# Autodesk Inventor assembly: robot_arm
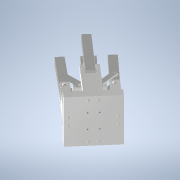
[picture p0: Inventor's stored thumbnail of the model, 180x180]
Saved by Autodesk Inventor 2021 (Build 250183000, 183)
## iProperties
Created: 2021-10-07
Part Number: robot_arm
Document SubType Name: Assembly
Designer: ryusei
Author: ryusei
## Documents named in this file (13)
- C:\Users\ryusei\Documents\Inventor\robot_design3\試作品1号\robot_arm.iam
- C:\Users\ryusei\Documents\Inventor\robot_design3\試作品1号\部品\土台.ipt
- C:\Users\ryusei\Documents\Inventor\robot_design3\試作品1号\部品\アーム支え.ipt
- C:\Users\ryusei\Documents\Inventor\robot_design3\試作品1号\部品\MF63ZZ_ベアリング.ipt
- C:\Users\ryusei\Documents\Inventor\robot_design3\試作品1号\部品\ステンレス平行ピンΦ3h7_20.ipt
- C:\Users\ryusei\Documents\Inventor\robot_design3\試作品1号\部品\シリンダ固定.ipt
- C:\Users\ryusei\Documents\Inventor\robot_design3\試作品1号\部品\シリンダ先端パーツ.ipt
- C:\Users\ryusei\Documents\Inventor\robot_design3\試作品1号\部品\アーム10×10×60.ipt
- C:\Users\ryusei\Documents\Inventor\robot_design3\試作品1号\部品\ステンレス平行ピンΦ3h7_16.ipt
- C:\Users\ryusei\Documents\Inventor\robot_design3\試作品1号\MBDA6×15_シリンダコガネイ\伸びるやつ１.ipt
- C:\Users\ryusei\Documents\Inventor\robot_design3\試作品1号\MBDA6×15_シリンダコガネイ\伸びるやつ2.ipt
- C:\Users\ryusei\Documents\Inventor\robot_design3\試作品1号\MBDA6×15_シリンダコガネイ\本体.ipt
- C:\Users\ryusei\Documents\Inventor\robot_design3\試作品1号\部品\リンク26×6×2.ipt
## Components (59 placed, 12 different names)
1. 土台:1 — 挿入:17, 挿入:18, 挿入:21, 挿入:22, 角度:1, 挿入:56, 挿入:57, 挿入:58, 挿入:59, 挿入:60, 挿入:61, 挿入:62, 挿入:63, 挿入:64, 挿入:65, 挿入:66, 挿入:67, 挿入:68, 挿入:69, 挿入:70, 挿入:71, 挿入:72, 挿入:73
2. アーム支え:1 — 挿入:9, 挿入:10, 挿入:62, 挿入:63, 挿入:72, 挿入:73
3. アーム支え:2 — 挿入:11, 挿入:12, 挿入:56, 挿入:57, 挿入:60, 挿入:61, 挿入:66, 挿入:67
4. アーム支え:3 — 挿入:13, 挿入:14, 挿入:58, 挿入:59, 挿入:68, 挿入:69
5. アーム支え:4 — 挿入:15, 挿入:16, 挿入:64, 挿入:65, 挿入:70, 挿入:71
6. MF63ZZ_ベアリング:1 — 挿入:15
7. MF63ZZ_ベアリング:2 — 挿入:13, メイト:3
8. MF63ZZ_ベアリング:3 — 挿入:10
9. MF63ZZ_ベアリング:4 — 挿入:12
10. MF63ZZ_ベアリング:5 — 挿入:16, メイト:18
11. MF63ZZ_ベアリング:6 — 挿入:11, メイト:4
12. MF63ZZ_ベアリング:7 — 挿入:14
13. MF63ZZ_ベアリング:8 — 挿入:9, メイト:2
14. ステンレス平行ピンΦ3h7_20:1 — メイト:4, メイト:8
15. ステンレス平行ピンΦ3h7_20:2 — メイト:3, メイト:5
16. ステンレス平行ピンΦ3h7_20:3 — メイト:2, メイト:7
17. シリンダ固定:1 — 挿入:17, 挿入:18
18. シリンダ固定:2 — 挿入:21, 挿入:22, 挿入:44, 挿入:45
19. アーム10×10×60:1 — メイト:8, 挿入:40, 挿入:41
20. アーム10×10×60:2 — メイト:7, 挿入:34, 挿入:35
21. アーム10×10×60:3 — メイト:5, 挿入:38, 挿入:39
22. アーム10×10×60:4 — 挿入:36, 挿入:37, メイト:19
23. MF63ZZ_ベアリング:17 — 挿入:40, メイト:12
24. MF63ZZ_ベアリング:18 — 挿入:41
25. MF63ZZ_ベアリング:19 — 挿入:36, メイト:9
26. MF63ZZ_ベアリング:20 — 挿入:37
27. MF63ZZ_ベアリング:21 — 挿入:38, メイト:10
28. MF63ZZ_ベアリング:22 — 挿入:39
29. MF63ZZ_ベアリング:23 — 挿入:35
30. MF63ZZ_ベアリング:24 — 挿入:34, メイト:11
31. ステンレス平行ピンΦ3h7_16:3 — メイト:12, 挿入:86, 挿入:99
32. ステンレス平行ピンΦ3h7_16:5 — メイト:11, 挿入:96, 挿入:101
33. ステンレス平行ピンΦ3h7_16:6 — メイト:9, 挿入:93, 挿入:95
34. ステンレス平行ピンΦ3h7_16:7 — メイト:10, 挿入:89, 挿入:91
35. シリンダ先端パーツ:1 — 角度:1, 挿入:46, 挿入:47, 挿入:48, 挿入:49, 挿入:50, 挿入:51, 挿入:52, 挿入:53
36. 伸びるやつ１:1
37. 伸びるやつ2:1
38. 本体:1 — 挿入:44, 挿入:45
39. MF63ZZ_ベアリング:25 — 挿入:49, メイト:14
40. MF63ZZ_ベアリング:26 — 挿入:48
41. MF63ZZ_ベアリング:27 — 挿入:47
42. MF63ZZ_ベアリング:28 — 挿入:46, メイト:16
43. MF63ZZ_ベアリング:29 — 挿入:50, メイト:15
44. MF63ZZ_ベアリング:30 — 挿入:51
45. MF63ZZ_ベアリング:31 — 挿入:52, メイト:17
46. MF63ZZ_ベアリング:32 — 挿入:53
47. ステンレス平行ピンΦ3h7_16:8 — メイト:16, 挿入:97, 挿入:100
48. ステンレス平行ピンΦ3h7_16:9 — メイト:15, 挿入:88, 挿入:90
49. ステンレス平行ピンΦ3h7_16:11 — メイト:14, 挿入:87, 挿入:98
50. ステンレス平行ピンΦ3h7_16:12 — メイト:17, 挿入:92, 挿入:94
51. ステンレス平行ピンΦ3h7_20:4 — メイト:18, メイト:19
52. リンク26×6×2:1 — 挿入:92, 挿入:93
53. リンク26×6×2:2 — 挿入:100, 挿入:101
54. リンク26×6×2:3 — 挿入:98, 挿入:99
55. リンク26×6×2:4 — 挿入:96, 挿入:97
56. リンク26×6×2:5 — 挿入:94, 挿入:95
57. リンク26×6×2:6 — 挿入:90, 挿入:91
58. リンク26×6×2:7 — 挿入:88, 挿入:89
59. リンク26×6×2:8 — 挿入:86, 挿入:87
## Relationships (84: Insert 66, Mate 17, Angle 1)
- 挿入:9 [Insert]: アーム支え:1 ↔ MF63ZZ_ベアリング:8
- 挿入:10 [Insert]: アーム支え:1 ↔ MF63ZZ_ベアリング:3
- 挿入:11 [Insert]: アーム支え:2 ↔ MF63ZZ_ベアリング:6
- 挿入:12 [Insert]: アーム支え:2 ↔ MF63ZZ_ベアリング:4
- 挿入:13 [Insert]: アーム支え:3 ↔ MF63ZZ_ベアリング:2
- 挿入:14 [Insert]: アーム支え:3 ↔ MF63ZZ_ベアリング:7
- 挿入:15 [Insert]: アーム支え:4 ↔ MF63ZZ_ベアリング:1
- 挿入:16 [Insert]: アーム支え:4 ↔ MF63ZZ_ベアリング:5
- メイト:2 [Mate]: MF63ZZ_ベアリング:8 ↔ ステンレス平行ピンΦ3h7_20:3
- メイト:3 [Mate]: MF63ZZ_ベアリング:2 ↔ ステンレス平行ピンΦ3h7_20:2
- メイト:4 [Mate]: MF63ZZ_ベアリング:6 ↔ ステンレス平行ピンΦ3h7_20:1
- 挿入:17 [Insert]: 土台:1 ↔ シリンダ固定:1
- 挿入:18 [Insert]: 土台:1 ↔ シリンダ固定:1
- 挿入:21 [Insert]: 土台:1 ↔ シリンダ固定:2
- 挿入:22 [Insert]: 土台:1 ↔ シリンダ固定:2
- メイト:5 [Mate]: ステンレス平行ピンΦ3h7_20:2 ↔ アーム10×10×60:3
- メイト:7 [Mate]: ステンレス平行ピンΦ3h7_20:3 ↔ アーム10×10×60:2
- メイト:8 [Mate]: ステンレス平行ピンΦ3h7_20:1 ↔ アーム10×10×60:1
- 挿入:34 [Insert]: アーム10×10×60:2 ↔ MF63ZZ_ベアリング:24
- 挿入:35 [Insert]: アーム10×10×60:2 ↔ MF63ZZ_ベアリング:23
- 挿入:36 [Insert]: アーム10×10×60:4 ↔ MF63ZZ_ベアリング:19
- 挿入:37 [Insert]: アーム10×10×60:4 ↔ MF63ZZ_ベアリング:20
- 挿入:38 [Insert]: アーム10×10×60:3 ↔ MF63ZZ_ベアリング:21
- 挿入:39 [Insert]: アーム10×10×60:3 ↔ MF63ZZ_ベアリング:22
- 挿入:40 [Insert]: アーム10×10×60:1 ↔ MF63ZZ_ベアリング:17
- 挿入:41 [Insert]: アーム10×10×60:1 ↔ MF63ZZ_ベアリング:18
- メイト:9 [Mate]: MF63ZZ_ベアリング:19 ↔ ステンレス平行ピンΦ3h7_16:6
- メイト:10 [Mate]: MF63ZZ_ベアリング:21 ↔ ステンレス平行ピンΦ3h7_16:7
- メイト:11 [Mate]: MF63ZZ_ベアリング:24 ↔ ステンレス平行ピンΦ3h7_16:5
- メイト:12 [Mate]: MF63ZZ_ベアリング:17 ↔ ステンレス平行ピンΦ3h7_16:3
- [Insert]: 伸びるやつ１:1 ↔ 伸びるやつ2:1
- [Mate]: 伸びるやつ１:1 ↔ 本体:1
- [Insert]: シリンダ先端パーツ:1 ↔ 伸びるやつ１:1
- 挿入:44 [Insert]: シリンダ固定:2 ↔ 本体:1
- 挿入:45 [Insert]: シリンダ固定:2 ↔ 本体:1
- 角度:1 [Angle] (0 deg): 土台:1 ↔ シリンダ先端パーツ:1
- 挿入:46 [Insert]: シリンダ先端パーツ:1 ↔ MF63ZZ_ベアリング:28
- 挿入:47 [Insert]: シリンダ先端パーツ:1 ↔ MF63ZZ_ベアリング:27
- 挿入:48 [Insert]: シリンダ先端パーツ:1 ↔ MF63ZZ_ベアリング:26
- 挿入:49 [Insert]: シリンダ先端パーツ:1 ↔ MF63ZZ_ベアリング:25
- 挿入:50 [Insert]: シリンダ先端パーツ:1 ↔ MF63ZZ_ベアリング:29
- 挿入:51 [Insert]: シリンダ先端パーツ:1 ↔ MF63ZZ_ベアリング:30
- 挿入:52 [Insert]: シリンダ先端パーツ:1 ↔ MF63ZZ_ベアリング:31
- 挿入:53 [Insert]: シリンダ先端パーツ:1 ↔ MF63ZZ_ベアリング:32
- メイト:14 [Mate]: MF63ZZ_ベアリング:25 ↔ ステンレス平行ピンΦ3h7_16:11
- メイト:15 [Mate]: MF63ZZ_ベアリング:29 ↔ ステンレス平行ピンΦ3h7_16:9
- メイト:16 [Mate]: MF63ZZ_ベアリング:28 ↔ ステンレス平行ピンΦ3h7_16:8
- メイト:17 [Mate]: MF63ZZ_ベアリング:31 ↔ ステンレス平行ピンΦ3h7_16:12
- 挿入:56 [Insert]: 土台:1 ↔ アーム支え:2
- 挿入:57 [Insert]: 土台:1 ↔ アーム支え:2
- 挿入:58 [Insert]: 土台:1 ↔ アーム支え:3
- 挿入:59 [Insert]: 土台:1 ↔ アーム支え:3
- 挿入:60 [Insert]: 土台:1 ↔ アーム支え:2
- 挿入:61 [Insert]: 土台:1 ↔ アーム支え:2
- 挿入:62 [Insert]: 土台:1 ↔ アーム支え:1
- 挿入:63 [Insert]: 土台:1 ↔ アーム支え:1
- 挿入:64 [Insert]: 土台:1 ↔ アーム支え:4
- 挿入:65 [Insert]: 土台:1 ↔ アーム支え:4
- 挿入:66 [Insert]: 土台:1 ↔ アーム支え:2
- 挿入:67 [Insert]: 土台:1 ↔ アーム支え:2
- 挿入:68 [Insert]: 土台:1 ↔ アーム支え:3
- 挿入:69 [Insert]: 土台:1 ↔ アーム支え:3
- 挿入:70 [Insert]: 土台:1 ↔ アーム支え:4
- 挿入:71 [Insert]: 土台:1 ↔ アーム支え:4
- 挿入:72 [Insert]: 土台:1 ↔ アーム支え:1
- 挿入:73 [Insert]: 土台:1 ↔ アーム支え:1
- メイト:18 [Mate]: MF63ZZ_ベアリング:5 ↔ ステンレス平行ピンΦ3h7_20:4
- メイト:19 [Mate]: アーム10×10×60:4 ↔ ステンレス平行ピンΦ3h7_20:4
- 挿入:86 [Insert]: ステンレス平行ピンΦ3h7_16:3 ↔ リンク26×6×2:8
- 挿入:87 [Insert]: ステンレス平行ピンΦ3h7_16:11 ↔ リンク26×6×2:8
- 挿入:88 [Insert]: ステンレス平行ピンΦ3h7_16:9 ↔ リンク26×6×2:7
- 挿入:89 [Insert]: ステンレス平行ピンΦ3h7_16:7 ↔ リンク26×6×2:7
- 挿入:90 [Insert]: ステンレス平行ピンΦ3h7_16:9 ↔ リンク26×6×2:6
- 挿入:91 [Insert]: ステンレス平行ピンΦ3h7_16:7 ↔ リンク26×6×2:6
- 挿入:92 [Insert]: ステンレス平行ピンΦ3h7_16:12 ↔ リンク26×6×2:1
- 挿入:93 [Insert]: ステンレス平行ピンΦ3h7_16:6 ↔ リンク26×6×2:1
- 挿入:94 [Insert]: ステンレス平行ピンΦ3h7_16:12 ↔ リンク26×6×2:5
- 挿入:95 [Insert]: ステンレス平行ピンΦ3h7_16:6 ↔ リンク26×6×2:5
- 挿入:96 [Insert]: ステンレス平行ピンΦ3h7_16:5 ↔ リンク26×6×2:4
- 挿入:97 [Insert]: ステンレス平行ピンΦ3h7_16:8 ↔ リンク26×6×2:4
- 挿入:98 [Insert]: ステンレス平行ピンΦ3h7_16:11 ↔ リンク26×6×2:3
- 挿入:99 [Insert]: ステンレス平行ピンΦ3h7_16:3 ↔ リンク26×6×2:3
- 挿入:100 [Insert]: ステンレス平行ピンΦ3h7_16:8 ↔ リンク26×6×2:2
- 挿入:101 [Insert]: ステンレス平行ピンΦ3h7_16:5 ↔ リンク26×6×2:2
